# Autodesk Inventor assembly: A_beam_end_mount
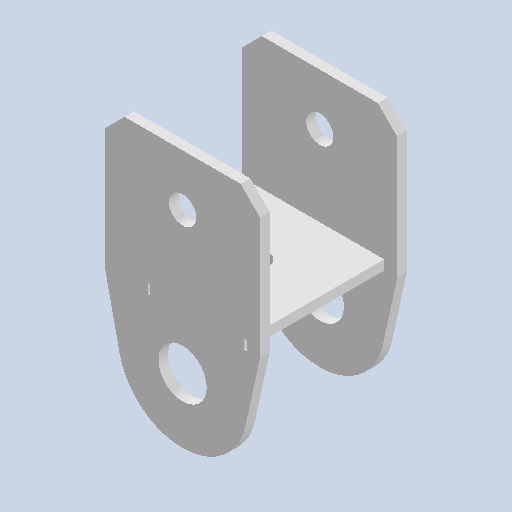
[picture p0: Inventor's stored thumbnail of the model, 512x512]
Saved by Autodesk Inventor 2025.2 (Build 292293000, 293)
## iProperties
Created: 2025-05-02
Part Number: A_beam_end_mount
Document SubType Name: Assembly
Designer: Caspe
Author: Caspe
## Documents named in this file (3)
- C:\Users\Caspe\Documents\Semester 8\Project\Anomaly_Detection\Mechanical_Project\Inventor_project\A_beam_end_mount.iam
- C:\Users\Caspe\Documents\Semester 8\Project\Anomaly_Detection\Mechanical_Project\Inventor_project\A_beam_end_mount_1.ipt
- C:\Users\Caspe\Documents\Semester 8\Project\Anomaly_Detection\Mechanical_Project\Inventor_project\A_beam_end_mount_2.ipt
## Components (3 placed, 2 different names)
1. A_beam_end_mount_1:1 — Mate:1, Mate:2, Mate:3, Mate:4
2. A_beam_end_mount_2:1 — Mate:3, Mate:4
3. A_beam_end_mount_2:2 — Mate:1, Mate:2
## Relationships (4: Mate 4)
- Mate:1: A_beam_end_mount_1:1 ↔ A_beam_end_mount_2:2
- Mate:2: A_beam_end_mount_1:1 ↔ A_beam_end_mount_2:2
- Mate:3: A_beam_end_mount_1:1 ↔ A_beam_end_mount_2:1
- Mate:4: A_beam_end_mount_1:1 ↔ A_beam_end_mount_2:1
